# Autodesk Inventor assembly: 2AM-17-A-5200 - claw
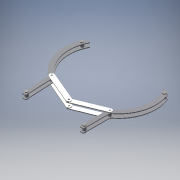
[picture p0: Inventor's stored thumbnail of the model, 180x180]
Saved by Autodesk Inventor 2017 (Build 210142000, 142)
## iProperties
Created: 2017-12-27
Part Number: 2AM-17-A-5200 - claw
Document SubType Name: Assembly
Designer: Micah
Author: Micah
## Documents named in this file (5)
- C:\Users\Micah\Desktop\inventor\CADathon-2017\2AM-17-A-0200 - Smokestack Elevator\2AM-17-A-5200 - claw.iam
- C:\Users\Micah\Desktop\inventor\CADathon-2017\2AM-17-A-0200 - Smokestack Elevator\2AM-17-A-6200 - claw arm.iam
- C:\Users\Micah\Documents\Inventor\Content Center Files\R2017\en-US\AS 2465(2)\AS 2465 - 1_4 x 1  UNC.ipt
- C:\Users\Micah\Documents\Inventor\Content Center Files\R2017\en-US\AS 2465(3)\AS 2465 - 1_4  UNC(2).ipt
- C:\Users\Micah\Desktop\inventor\CADathon-2017\2AM-17-A-0200 - Smokestack Elevator\2AM-17-P-5204 - links.ipt
## Components (10 placed, 4 different names)
1. 2AM-17-A-6200 - claw arm:1 [sub-assembly] — Rotational:3, Rotational:4, Mate:3
2. 2AM-17-A-6200 - claw arm:2 [sub-assembly] — Insert:1, Insert:3, Insert:4, Insert:6, Rotational:1, Rotational:2, Mate:3
3. AS 2465 - Inch 1/4 x 1  UNC:1 — Insert:1
4. AS 2465 - Inch 1/4 x 1  UNC:3 — Insert:3
5. AS 2465 (Unified hexagon bolts, screws and nuts (UNC and UNF threads) - Inch 1/4  UNC:1 — Insert:4
6. AS 2465 (Unified hexagon bolts, screws and nuts (UNC and UNF threads) - Inch 1/4  UNC:3 — Insert:6
7. 2AM-17-P-5204 - links:1 — Rotational:1, Mate:1
8. 2AM-17-P-5204 - links:2 — Rotational:2, Mate:2
9. 2AM-17-P-5204 - links:3 — Rotational:4, Mate:1
10. 2AM-17-P-5204 - links:4 — Rotational:3, Mate:2
## Relationships (11: Insert 4, RevoluteJoint 4, Mate 3)
- Insert:1: 2AM-17-A-6200 - claw arm:2 ↔ AS 2465 - Inch 1/4 x 1  UNC:1
- Insert:3: 2AM-17-A-6200 - claw arm:2 ↔ AS 2465 - Inch 1/4 x 1  UNC:3
- Insert:4: 2AM-17-A-6200 - claw arm:2 ↔ AS 2465 (Unified hexagon bolts, screws and nuts (UNC and UNF threads) - Inch 1/4  UNC:1
- Insert:6: 2AM-17-A-6200 - claw arm:2 ↔ AS 2465 (Unified hexagon bolts, screws and nuts (UNC and UNF threads) - Inch 1/4  UNC:3
- Rotational:1 [RevoluteJoint]: 2AM-17-A-6200 - claw arm:2 ↔ 2AM-17-P-5204 - links:1
- Rotational:2 [RevoluteJoint]: 2AM-17-A-6200 - claw arm:2 ↔ 2AM-17-P-5204 - links:2
- Rotational:3 [RevoluteJoint]: 2AM-17-A-6200 - claw arm:1 ↔ 2AM-17-P-5204 - links:4
- Rotational:4 [RevoluteJoint]: 2AM-17-A-6200 - claw arm:1 ↔ 2AM-17-P-5204 - links:3
- Mate:1: 2AM-17-P-5204 - links:1 ↔ 2AM-17-P-5204 - links:3
- Mate:2: 2AM-17-P-5204 - links:2 ↔ 2AM-17-P-5204 - links:4
- Mate:3: 2AM-17-A-6200 - claw arm:1 ↔ 2AM-17-A-6200 - claw arm:2
